# Autodesk Inventor assembly: ClawLauncher
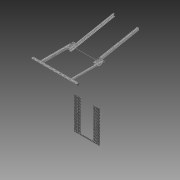
[picture p0: Inventor's stored thumbnail of the model, 180x180]
Saved by Autodesk Inventor 2015 (Build 190159000, 159)
## iProperties
Created: 2016-09-16
Part Number: ClawLauncher
Document SubType Name: Assembly
Designer: wangl
Author: wangl
## Documents named in this file (17)
- C:\Users\Leo\Google Drive\StarStuckProject\Starstruck\Prototypes\ClawLauncher2.iam
- C:\Users\Leo\Google Drive\StarStuckProject\Starstruck\Imported Components\C-Channel 1x2x1x35\C-Channel 1x2x1x35 2.0.ipt
- C:\Users\Leo\Google Drive\StarStuckProject\Starstruck\Imported Components\Chasis Rail 2x1x25\Chasis Rail 2x1x25.ipt
- C:\Users\Leo\Google Drive\StarStuckProject\Starstruck\Imported Components\Angle 2x2x35\Angle 2x2x35.ipt
- C:\Users\Leo\Google Drive\StarStuckProject\Starstruck\Imported Components\Large Screw .500In\Large Screw .500In.ipt
- C:\Users\Leo\Google Drive\StarStuckProject\Starstruck\Imported Components\Flat Bearing\Flat Bearing.ipt
- C:\Users\Leo\Google Drive\StarStuckProject\Starstruck\Imported Components\Large Screw .25In\Large Screw .25In.ipt
- C:\Users\Leo\Google Drive\StarStuckProject\Starstruck\Imported Components\Regular Nut\Regular Nut.ipt
- C:\Users\Leo\Google Drive\StarStuckProject\Starstruck\Imported Components\Axle 12in\Axle 12in.ipt
- C:\Users\Leo\Google Drive\StarStuckProject\Starstruck\Imported Components\Shaft Collar\Shaft Collar.ipt
- C:\Users\Leo\Google Drive\StarStuckProject\Starstruck\Imported Components\60T HS Gear\60T HS Gear.ipt
- C:\Users\Leo\Google Drive\StarStuckProject\Starstruck\Imported Components\HS Gear Metal Insert\HS Gear Metal Insert.ipt
- C:\Users\Leo\Google Drive\StarStuckProject\Starstruck\Imported Components\Large 1.00in Screw\Large 1.00in Screw.ipt
- C:\Users\Leo\Google Drive\StarStuckProject\Starstruck\Imported Components\12T HS Gear\12T HS Gear.ipt
- C:\Users\Leo\Google Drive\StarStuckProject\Starstruck\Imported Components\Small Screw .50In\Small Screw .50In.ipt
- C:\Users\Leo\Google Drive\StarStuckProject\Starstruck\Imported Components\Plate 5x25\Plate 5x25.ipt
- C:\Users\Leo\Google Drive\StarStuckProject\Starstruck\VEX Parts\Structure\Metal\Bars\1x20 Bar.ipt
## Components (54 placed, 16 different names)
1. C-Channel 1x2x1x35 2.0:1 — Mate:44, Tangent:29, Tangent:30, Tangent:32, Tangent:37, Mate:45, Mate:46
2. Chasis Rail 2x1x25:1 — Flush:4, Mate:4, Flush:6, Mate:13, Tangent:13, Tangent:14, Tangent:15, Tangent:16, Mate:16, Mate:17, Mate:23, Mate:24, Tangent:26, Mate:49, Mate:61, Mate:62, Tangent:56, Tangent:57, Tangent:58, Tangent:59
3. Chasis Rail 2x1x25:2 — Mate:3, Flush:3, Flush:5, Mate:5, Mate:6, Mate:7, Tangent:7, Tangent:8, Tangent:9, Tangent:10, Mate:14, Mate:15, Mate:74, Mate:73
4. C-Channel 1x2x1x35 2.0:2 — Mate:43, Tangent:33, Tangent:34, Tangent:35, Tangent:36, Mate:47, Mate:48
5. Angle 2x2x35:2 — Mate:3, Flush:3, Flush:4, Mate:4, Flush:5, Flush:6, Tangent:1, Tangent:2, Tangent:3, Tangent:4, Mate:18, Mate:19, Mate:20, Mate:21, Tangent:23, Tangent:24, Tangent:25
6. Flat Bearing:1 — Mate:11, Mate:12, Tangent:11, Tangent:12, Mate:13
7. Flat Bearing:2 — Mate:5, Mate:8, Mate:9, Tangent:5, Tangent:6, Insert:1, Insert:3
8. Large Screw .25In:1 — Mate:7, Tangent:1, Tangent:3, Tangent:21
9. Large Screw .25In:2 — Mate:6, Tangent:2, Tangent:4, Tangent:22
10. Large Screw .500In:1 — Mate:8, Tangent:6, Tangent:8, Tangent:10, Tangent:20
11. Large Screw .500In:2 — Mate:9, Tangent:5, Tangent:7, Tangent:9, Tangent:19
12. Large Screw .500In:3 — Mate:12, Tangent:12, Tangent:14, Tangent:15, Tangent:17
13. Large Screw .500In:4 — Mate:11, Tangent:11, Tangent:13, Tangent:16, Tangent:18
14. Regular Nut:1 — Mate:15, Tangent:19
15. Regular Nut:2 — Mate:14, Tangent:20
16. Regular Nut:3 — Mate:16, Tangent:18
17. Regular Nut:4 — Mate:17, Tangent:17
18. Regular Nut:5 — Mate:18, Tangent:21
19. Regular Nut:6 — Mate:19, Tangent:22
20. Regular Nut:7 — Mate:20, Tangent:28
21. Regular Nut:8 — Mate:21, Tangent:27
22. Large Screw .25In:3 — Mate:24, Tangent:23, Tangent:26, Tangent:28
23. Large Screw .25In:4 — Mate:23, Tangent:24, Tangent:25, Tangent:27
24. Axle 12in:1 — Insert:1, Insert:2, Mate:37, Mate:38, Mate:39, Mate:40
25. Shaft Collar:1 — Insert:2, Mate:42, Insert:9
26. Shaft Collar:2 — Insert:3, Mate:41, Insert:8
27. 60T HS Gear:1 — Mate:25, Mate:27, Mate:28, Mate:29, Mate:30, Mate:31, Insert:6, Insert:7, Mate:44
28. 60T HS Gear:2 — Mate:26, Mate:32, Mate:33, Mate:34, Mate:35, Mate:36, Insert:4, Insert:5, Mate:43
29. HS Gear Metal Insert:1 — Mate:26, Mate:33, Mate:35, Mate:39, Mate:40, Mate:41
30. HS Gear Metal Insert:2 — Mate:32, Mate:34, Mate:36
31. HS Gear Metal Insert:3 — Mate:25, Mate:27, Mate:28, Mate:37, Mate:38
32. HS Gear Metal Insert:4 — Mate:29, Mate:30, Mate:31, Mate:42
33. Large 1.00in Screw:1 — Insert:4, Tangent:33, Tangent:36, Tangent:41
34. Large 1.00in Screw:2 — Insert:5, Tangent:34, Tangent:35, Tangent:40
35. Large 1.00in Screw:3 — Insert:7, Tangent:29, Tangent:32, Tangent:39
36. Large 1.00in Screw:4 — Insert:6, Tangent:30, Tangent:37, Tangent:38
37. Regular Nut:9 — Mate:48, Tangent:41
38. Regular Nut:10 — Mate:45, Tangent:38
39. Regular Nut:11 — Mate:47, Tangent:40
40. Regular Nut:12 — Mate:46, Tangent:39
41. Flat Bearing:3 — Mate:49, Mate:53, Mate:54, Tangent:42, Tangent:43
42. Large Screw .500In:7 — Mate:53, Tangent:42, Tangent:56, Tangent:57, Tangent:61
43. Large Screw .500In:8 — Mate:54, Tangent:43, Tangent:58, Tangent:59, Tangent:60
44. 12T HS Gear:1 — Mate:64
45. Shaft Collar:3 — Mate:64
46. Shaft Collar:4 — Insert:9
47. Shaft Collar:5 — Insert:8
48. Regular Nut:15 — Mate:61, Tangent:61
49. Regular Nut:16 — Mate:62, Tangent:60
50. Small Screw .50In:1 — Mate:73
51. Small Screw .50In:2 — Mate:74
52. Plate 5x25:1 — Mate:83, Flush:11, Flush:12
53. Plate 5x25:2 — Mate:82, Flush:13, Flush:14
54. 1x20 Bar:1 — Mate:82, Mate:83, Flush:11, Flush:12, Flush:13, Flush:14
## Relationships (119: Mate 54, Tangent 48, Insert 9, Flush 8)
- Mate:3: Chasis Rail 2x1x25:2 ↔ Angle 2x2x35:2
- Flush:3: Chasis Rail 2x1x25:2 ↔ Angle 2x2x35:2
- Flush:4: Chasis Rail 2x1x25:1 ↔ Angle 2x2x35:2
- Mate:4: Chasis Rail 2x1x25:1 ↔ Angle 2x2x35:2
- Flush:5: Chasis Rail 2x1x25:2 ↔ Angle 2x2x35:2
- Flush:6: Chasis Rail 2x1x25:1 ↔ Angle 2x2x35:2
- Mate:5: Chasis Rail 2x1x25:2 ↔ Flat Bearing:2
- Mate:6: Chasis Rail 2x1x25:2 ↔ Large Screw .25In:2
- Mate:7: Chasis Rail 2x1x25:2 ↔ Large Screw .25In:1
- Tangent:1: Angle 2x2x35:2 ↔ Large Screw .25In:1
- Tangent:2: Angle 2x2x35:2 ↔ Large Screw .25In:2
- Tangent:3: Angle 2x2x35:2 ↔ Large Screw .25In:1
- Tangent:4: Angle 2x2x35:2 ↔ Large Screw .25In:2
- Mate:8: Flat Bearing:2 ↔ Large Screw .500In:1
- Mate:9: Flat Bearing:2 ↔ Large Screw .500In:2
- Tangent:5: Flat Bearing:2 ↔ Large Screw .500In:2
- Tangent:6: Flat Bearing:2 ↔ Large Screw .500In:1
- Tangent:7: Chasis Rail 2x1x25:2 ↔ Large Screw .500In:2
- Tangent:8: Chasis Rail 2x1x25:2 ↔ Large Screw .500In:1
- Tangent:9: Chasis Rail 2x1x25:2 ↔ Large Screw .500In:2
- Tangent:10: Chasis Rail 2x1x25:2 ↔ Large Screw .500In:1
- Mate:11: Flat Bearing:1 ↔ Large Screw .500In:4
- Mate:12: Flat Bearing:1 ↔ Large Screw .500In:3
- Tangent:11: Flat Bearing:1 ↔ Large Screw .500In:4
- Tangent:12: Flat Bearing:1 ↔ Large Screw .500In:3
- Mate:13: Chasis Rail 2x1x25:1 ↔ Flat Bearing:1
- Tangent:13: Chasis Rail 2x1x25:1 ↔ Large Screw .500In:4
- Tangent:14: Chasis Rail 2x1x25:1 ↔ Large Screw .500In:3
- Tangent:15: Chasis Rail 2x1x25:1 ↔ Large Screw .500In:3
- Tangent:16: Chasis Rail 2x1x25:1 ↔ Large Screw .500In:4
- Mate:14: Chasis Rail 2x1x25:2 ↔ Regular Nut:2
- Mate:15: Chasis Rail 2x1x25:2 ↔ Regular Nut:1
- Mate:16: Chasis Rail 2x1x25:1 ↔ Regular Nut:3
- Mate:17: Chasis Rail 2x1x25:1 ↔ Regular Nut:4
- Tangent:17: Large Screw .500In:3 ↔ Regular Nut:4
- Tangent:18: Large Screw .500In:4 ↔ Regular Nut:3
- Tangent:19: Large Screw .500In:2 ↔ Regular Nut:1
- Tangent:20: Large Screw .500In:1 ↔ Regular Nut:2
- Mate:18: Angle 2x2x35:2 ↔ Regular Nut:5
- Mate:19: Angle 2x2x35:2 ↔ Regular Nut:6
- Mate:20: Angle 2x2x35:2 ↔ Regular Nut:7
- Mate:21: Angle 2x2x35:2 ↔ Regular Nut:8
- Tangent:21: Large Screw .25In:1 ↔ Regular Nut:5
- Tangent:22: Large Screw .25In:2 ↔ Regular Nut:6
- Mate:23: Chasis Rail 2x1x25:1 ↔ Large Screw .25In:4
- Mate:24: Chasis Rail 2x1x25:1 ↔ Large Screw .25In:3
- Tangent:23: Angle 2x2x35:2 ↔ Large Screw .25In:3
- Tangent:24: Angle 2x2x35:2 ↔ Large Screw .25In:4
- Tangent:25: Angle 2x2x35:2 ↔ Large Screw .25In:4
- Tangent:26: Chasis Rail 2x1x25:1 ↔ Large Screw .25In:3
- Tangent:27: Regular Nut:8 ↔ Large Screw .25In:4
- Tangent:28: Regular Nut:7 ↔ Large Screw .25In:3
- Insert:1: Flat Bearing:2 ↔ Axle 12in:1
- Insert:2 (7.62 mm): Axle 12in:1 ↔ Shaft Collar:1
- Insert:3 (7.62 mm): Flat Bearing:2 ↔ Shaft Collar:2
- Mate:25: 60T HS Gear:1 ↔ HS Gear Metal Insert:3
- Mate:26: 60T HS Gear:2 ↔ HS Gear Metal Insert:1
- Mate:27: 60T HS Gear:1 ↔ HS Gear Metal Insert:3
- Mate:28: 60T HS Gear:1 ↔ HS Gear Metal Insert:3
- Mate:29: 60T HS Gear:1 ↔ HS Gear Metal Insert:4
- Mate:30: 60T HS Gear:1 ↔ HS Gear Metal Insert:4
- Mate:31: 60T HS Gear:1 ↔ HS Gear Metal Insert:4
- Mate:32: 60T HS Gear:2 ↔ HS Gear Metal Insert:2
- Mate:33: 60T HS Gear:2 ↔ HS Gear Metal Insert:1
- Mate:34: 60T HS Gear:2 ↔ HS Gear Metal Insert:2
- Mate:35: 60T HS Gear:2 ↔ HS Gear Metal Insert:1
- Mate:36: 60T HS Gear:2 ↔ HS Gear Metal Insert:2
- Mate:37: Axle 12in:1 ↔ HS Gear Metal Insert:3
- Mate:38: Axle 12in:1 ↔ HS Gear Metal Insert:3
- Mate:39: Axle 12in:1 ↔ HS Gear Metal Insert:1
- Mate:40: Axle 12in:1 ↔ HS Gear Metal Insert:1
- Mate:41: Shaft Collar:2 ↔ HS Gear Metal Insert:1
- Mate:42: Shaft Collar:1 ↔ HS Gear Metal Insert:4
- Insert:4: 60T HS Gear:2 ↔ Large 1.00in Screw:1
- Insert:5: 60T HS Gear:2 ↔ Large 1.00in Screw:2
- Insert:6: 60T HS Gear:1 ↔ Large 1.00in Screw:4
- Insert:7: 60T HS Gear:1 ↔ Large 1.00in Screw:3
- Mate:43: C-Channel 1x2x1x35 2.0:2 ↔ 60T HS Gear:2
- Mate:44: C-Channel 1x2x1x35 2.0:1 ↔ 60T HS Gear:1
- Tangent:29: C-Channel 1x2x1x35 2.0:1 ↔ Large 1.00in Screw:3
- Tangent:30: C-Channel 1x2x1x35 2.0:1 ↔ Large 1.00in Screw:4
- Tangent:32: C-Channel 1x2x1x35 2.0:1 ↔ Large 1.00in Screw:3
- Tangent:33: C-Channel 1x2x1x35 2.0:2 ↔ Large 1.00in Screw:1
- Tangent:34: C-Channel 1x2x1x35 2.0:2 ↔ Large 1.00in Screw:2
- Tangent:35: C-Channel 1x2x1x35 2.0:2 ↔ Large 1.00in Screw:2
- Tangent:36: C-Channel 1x2x1x35 2.0:2 ↔ Large 1.00in Screw:1
- Tangent:37: C-Channel 1x2x1x35 2.0:1 ↔ Large 1.00in Screw:4
- Mate:45: C-Channel 1x2x1x35 2.0:1 ↔ Regular Nut:10
- Mate:46: C-Channel 1x2x1x35 2.0:1 ↔ Regular Nut:12
- Tangent:38: Large 1.00in Screw:4 ↔ Regular Nut:10
- Tangent:39: Large 1.00in Screw:3 ↔ Regular Nut:12
- Mate:47: C-Channel 1x2x1x35 2.0:2 ↔ Regular Nut:11
- Mate:48: C-Channel 1x2x1x35 2.0:2 ↔ Regular Nut:9
- Tangent:40: Large 1.00in Screw:2 ↔ Regular Nut:11
- Tangent:41: Large 1.00in Screw:1 ↔ Regular Nut:9
- Mate:49: Chasis Rail 2x1x25:1 ↔ Flat Bearing:3
- Mate:53: Flat Bearing:3 ↔ Large Screw .500In:7
- Mate:54: Flat Bearing:3 ↔ Large Screw .500In:8
- Tangent:42: Flat Bearing:3 ↔ Large Screw .500In:7
- Tangent:43: Flat Bearing:3 ↔ Large Screw .500In:8
- Insert:8 (20.32 mm): Shaft Collar:2 ↔ Shaft Collar:5
- Insert:9 (20.32 mm): Shaft Collar:1 ↔ Shaft Collar:4
- Mate:61: Chasis Rail 2x1x25:1 ↔ Regular Nut:15
- Mate:62: Chasis Rail 2x1x25:1 ↔ Regular Nut:16
- Mate:64: 12T HS Gear:1 ↔ Shaft Collar:3
- Tangent:56: Chasis Rail 2x1x25:1 ↔ Large Screw .500In:7
- Tangent:57: Chasis Rail 2x1x25:1 ↔ Large Screw .500In:7
- Tangent:58: Chasis Rail 2x1x25:1 ↔ Large Screw .500In:8
- Tangent:59: Chasis Rail 2x1x25:1 ↔ Large Screw .500In:8
- Tangent:60: Large Screw .500In:8 ↔ Regular Nut:16
- Tangent:61: Large Screw .500In:7 ↔ Regular Nut:15
- Mate:73: Chasis Rail 2x1x25:2 ↔ Small Screw .50In:1
- Mate:74: Chasis Rail 2x1x25:2 ↔ Small Screw .50In:2
- Mate:82: Plate 5x25:2 ↔ 1x20 Bar:1
- Mate:83: Plate 5x25:1 ↔ 1x20 Bar:1
- Flush:11: Plate 5x25:1 ↔ 1x20 Bar:1
- Flush:12: Plate 5x25:1 ↔ 1x20 Bar:1
- Flush:13: Plate 5x25:2 ↔ 1x20 Bar:1
- Flush:14: Plate 5x25:2 ↔ 1x20 Bar:1
